# Autodesk Inventor assembly: WemosLightSwitchV2
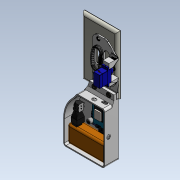
[picture p0: Inventor's stored thumbnail of the model, 180x180]
Saved by Autodesk Inventor 2020.2 (Build 242310000, 310)
## iProperties
Created: 2020-04-30
Part Number: WemosLightSwitchV2
Document SubType Name: Assembly
Designer: Haashim Rehan
Author: Haashim Rehan
## Documents named in this file (13)
- C:\Users\Dell\Documents\GitHub\Automatic-Light-Switch\CAD\WemosLightSwitchV2.iam
- C:\Users\Dell\Documents\GitHub\Automatic-Light-Switch\CAD\Light Switch Cover.ipt
- C:\Users\Dell\Documents\GitHub\Automatic-Light-Switch\CAD\WEMOS D1 mini.ipt
- C:\Users\Dell\Documents\GitHub\Automatic-Light-Switch\CAD\ble_switch_mount.ipt
- C:\Users\Dell\Documents\GitHub\Automatic-Light-Switch\CAD\Servo\microservoAssembly.iam
- C:\Users\Dell\Documents\GitHub\Automatic-Light-Switch\CAD\BatteryV1.ipt
- C:\Users\Dell\Documents\GitHub\Automatic-Light-Switch\CAD\BarrelJack.ipt
- C:\Users\Dell\Documents\Inventor\Content Center Files\R2020\en-US\HD00XX-M5\HD0028-M5x8.ipt
- C:\Users\Dell\Documents\Inventor\Content Center Files\R2020\en-US\HD00XX-M5\HD0012-M5.ipt
- C:\Users\Dell\Documents\GitHub\Automatic-Light-Switch\CAD\MainBaseV2.ipt
- C:\Users\Dell\Documents\GitHub\Automatic-Light-Switch\CAD\BatteryConnector.ipt
- C:\Users\Dell\Documents\GitHub\Automatic-Light-Switch\CAD\WemosCover.ipt
- C:\Users\Dell\Documents\GitHub\Automatic-Light-Switch\CAD\Buck Converter\LM2596 DC-DC StepDown Converter v2.iam
## Components (13 placed, 12 different names)
1. Light Switch Cover:1 — Mate:6, Mate:7, Mate:8
2. WEMOS D1 mini:2 — Mate:23, Mate:24, Flush:1
3. MainBaseV2:1 — Mate:4, Mate:5, Angle:1, Mate:6, Mate:7, Mate:8, Mate:9, Mate:10, Mate:11, Mate:12, Mate:13, Mate:14, Mate:15, Mate:16, Mate:20, Mate:21, Mate:22, Mate:23, Mate:24, Flush:1
4. microservoAssembly:1 [sub-assembly] — Mate:4, Mate:5, Angle:1
5. BatteryV1:1 — Mate:12, Mate:13
6. LM2596 DC-DC StepDown Converter v2:1 [sub-assembly]
7. BarrelJack:1 — Mate:17, Mate:18
8. ble_switch_mount:1
9. HD0028-M5x8:1 — Mate:11, Mate:14
10. HD0012-M5:1 — Mate:9, Mate:10
11. HD0028-M5x8:2 — Mate:15, Mate:16
12. BatteryConnector:1 — Mate:17, Mate:18
13. WemosCover:1 — Mate:20, Mate:21, Mate:22
## Relationships (22: Mate 20, Angle 1, Flush 1)
- Mate:4: MainBaseV2:1 ↔ microservoAssembly:1
- Mate:5: MainBaseV2:1 ↔ microservoAssembly:1
- Angle:1 (0 deg): MainBaseV2:1 ↔ microservoAssembly:1
- Mate:6: Light Switch Cover:1 ↔ MainBaseV2:1
- Mate:7: Light Switch Cover:1 ↔ MainBaseV2:1
- Mate:8: Light Switch Cover:1 ↔ MainBaseV2:1
- Mate:9: MainBaseV2:1 ↔ HD0012-M5:1
- Mate:10: MainBaseV2:1 ↔ HD0012-M5:1
- Mate:11: MainBaseV2:1 ↔ HD0028-M5x8:1
- Mate:12: MainBaseV2:1 ↔ BatteryV1:1
- Mate:13: MainBaseV2:1 ↔ BatteryV1:1
- Mate:14: MainBaseV2:1 ↔ HD0028-M5x8:1
- Mate:15: MainBaseV2:1 ↔ HD0028-M5x8:2
- Mate:16: MainBaseV2:1 ↔ HD0028-M5x8:2
- Mate:17: BarrelJack:1 ↔ BatteryConnector:1
- Mate:18: BarrelJack:1 ↔ BatteryConnector:1
- Mate:20 (0.25 mm): MainBaseV2:1 ↔ WemosCover:1
- Mate:21 (0.25 mm): MainBaseV2:1 ↔ WemosCover:1
- Mate:22 (0.5 mm): MainBaseV2:1 ↔ WemosCover:1
- Mate:23: WEMOS D1 mini:2 ↔ MainBaseV2:1
- Mate:24: WEMOS D1 mini:2 ↔ MainBaseV2:1
- Flush:1: WEMOS D1 mini:2 ↔ MainBaseV2:1
